# Autodesk Inventor assembly: Cottini lamp2
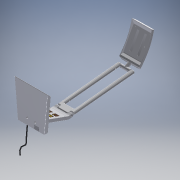
[picture p0: Inventor's stored thumbnail of the model, 180x180]
Saved by Autodesk Inventor 2016 (Build 200138000, 138)
## iProperties
Created: 2017-09-04
Part Number: Cottini lamp2
Document SubType Name: Assembly
Designer: Davide
Author: Davide
## Documents named in this file (22)
- C:\Users\Davide\Documents\Inventor\Cottini Lamp\Cottini lamp2.iam
- C:\Users\Davide\Documents\Inventor\Cottini Lamp\base bella.ipt
- C:\Users\Davide\Documents\Inventor\Cottini Lamp\perno bello.ipt
- C:\Users\Davide\Documents\Inventor\Cottini Lamp\USB Case.ipt
- C:\Users\Davide\Documents\Inventor\Cottini Lamp\cable.ipt
- C:\Users\Davide\Documents\Inventor\Cottini Lamp\tavolo.ipt
- C:\Users\Davide\Documents\Inventor\Cottini Lamp\primoblocco1.ipt
- C:\Users\Davide\Documents\Inventor\Cottini Lamp\placca.ipt
- C:\Users\Davide\Documents\Inventor\Content Center Files\R2016\en-US\AS 1427(03)\AS 1427 - M2 x 5(1).ipt
- C:\Users\Davide\Documents\Inventor\Cottini Lamp\Open_Book.ipt
- C:\Users\Davide\Documents\Inventor\Cottini Lamp\proiettore bello1.ipt
- C:\Users\Davide\Documents\Inventor\Cottini Lamp\astabella_lunga.ipt
- C:\Users\Davide\Documents\Inventor\Cottini Lamp\astabella_bassa.ipt
- C:\Users\Davide\Documents\Inventor\Content Center Files\R2016\en-US\AS 1112 (2)\AS 1112 - M4  Type 5.ipt
- C:\Users\Davide\Documents\Inventor\Content Center Files\R2016\en-US\AS 1427(05)\AS 1427 - M4 x 25(5) II.ipt
- C:\Users\Davide\Documents\Inventor\Content Center Files\R2016\en-US\AS 1420\AS 1420 - 1973 - M4 x 25.ipt
- C:\Users\Davide\Documents\Inventor\Content Center Files\R2016\en-US\AS 1112 (4)\AS 1112 - M4(2).ipt
- C:\Users\Davide\Documents\Inventor\Cottini Lamp\button1.ipt
- C:\Users\Davide\Documents\Inventor\Cottini Lamp\button2.ipt
- C:\Users\Davide\Documents\Inventor\Cottini Lamp\button3.ipt
- C:\Users\Davide\Documents\Inventor\Cottini Lamp\button4.ipt
- C:\Users\Davide\Documents\Inventor\Cottini Lamp\coperchietto.ipt
## Components (34 placed, 21 different names)
1. base bella:1 — Mate:47, Mate:49, Mate:50, Mate:51, Mate:79, Flush:1, Mate:80, Mate:94, Mate:95, Mate:96, Mate:110, Mate:112, Mate:209, Mate:210, Mate:211
2. perno bello:1 — Mate:147, Mate:148, Mate:153, Mate:173, Mate:175, Mate:178, Mate:180, Mate:182, Mate:183
3. USB Case:1 — Mate:79, Flush:1, Mate:80
4. cable:1 — Mate:112
5. tavolo:1 — Mate:94, Mate:146
6. primoblocco1:1 — Mate:95, Mate:96, Mate:138, Mate:139, Mate:155, Mate:160, Mate:161, Mate:164, Mate:165, Mate:166, Mate:167, Mate:188, Mate:207, Mate:208
7. placca:1 — Flush:6, Flush:7, Mate:192, Flush:12, Mate:199, Mate:200, Flush:13, Mate:201, Mate:202, Flush:14, Mate:203, Mate:204, Flush:15, Mate:205, Mate:206, Mate:207, Mate:208
8. Open_Book:1 — Mate:146
9. proiettore bello1:1 — Mate:147, Mate:148
10. astabella_lunga:1 — Mate:149, Mate:150, Mate:151, Mate:153, Mate:169, Mate:170, Mate:171, Mate:172
11. astabella_bassa:1 — Mate:149, Mate:150, Mate:151, Mate:155, Mate:168, Mate:185, Mate:187
12. button1:1 — Flush:12, Mate:199, Mate:200
13. button2:1 — Flush:13, Mate:201, Mate:202
14. button3:1 — Flush:14, Mate:203, Mate:204
15. button4:1 — Flush:15, Mate:205, Mate:206
16. coperchietto:1 — Mate:209, Mate:210, Mate:211, Mate:212, Mate:213, Flush:16, Flush:17
17. AS 1427 H - Metric M4 x 25:1 — Mate:47, Mate:51, Mate:158
18. AS 1427 H - Metric M4 x 25:2 — Mate:49, Mate:50, Mate:159
19. AS 1427 - Metric M2 x 5:2 — Mate:138, Flush:6, Mate:192
20. AS 1427 - Metric M2 x 5:3 — Mate:188
21. AS 1427 - Metric M2 x 5:6 — Mate:213, Flush:16
22. AS 1427 - Metric M2 x 5:7 — Mate:212, Flush:17
23. AS 1112 (2) - Metric M4  Type 5:1 — Mate:158, Mate:161
24. AS 1112 (2) - Metric M4  Type 5:2 — Mate:159, Mate:160
25. AS 1427 - Metric M2 x 5:4
26. AS 1427 - Metric M2 x 5:5 — Mate:139, Flush:7
27. AS 1420 - Metric M4 x 25:1 — Mate:164, Mate:167, Mate:184
28. AS 1420 - Metric M4 x 25:2 — Mate:165, Mate:166, Mate:168, Mate:186
29. AS 1420 - Metric M4 x 25:3 — Mate:169, Mate:170, Mate:175, Mate:178, Mate:179
30. AS 1420 - Metric M4 x 25:4 — Mate:171, Mate:172, Mate:173, Mate:181, Mate:182
31. AS 1112 (4) - Metric M4:1 — Mate:179, Mate:180
32. AS 1112 (4) - Metric M4:2 — Mate:181, Mate:183
33. AS 1112 (4) - Metric M4:3 — Mate:184, Mate:185
34. AS 1112 (4) - Metric M4:4 — Mate:186, Mate:187
## Relationships (74: Mate 65, Flush 9)
- Mate:47: base bella:1 ↔ AS 1427 H - Metric M4 x 25:1
- Mate:49: base bella:1 ↔ AS 1427 H - Metric M4 x 25:2
- Mate:50: base bella:1 ↔ AS 1427 H - Metric M4 x 25:2
- Mate:51: base bella:1 ↔ AS 1427 H - Metric M4 x 25:1
- Mate:79: base bella:1 ↔ USB Case:1
- Flush:1 (1 mm): base bella:1 ↔ USB Case:1
- Mate:80: base bella:1 ↔ USB Case:1
- Mate:94: base bella:1 ↔ tavolo:1
- Mate:95: base bella:1 ↔ primoblocco1:1
- Mate:96: base bella:1 ↔ primoblocco1:1
- Mate:110: base bella:1
- Mate:112: base bella:1 ↔ cable:1
- Mate:138: primoblocco1:1 ↔ AS 1427 - Metric M2 x 5:2
- Mate:139: primoblocco1:1 ↔ AS 1427 - Metric M2 x 5:5
- Flush:6: placca:1 ↔ AS 1427 - Metric M2 x 5:2
- Flush:7: placca:1 ↔ AS 1427 - Metric M2 x 5:5
- Mate:146: tavolo:1 ↔ Open_Book:1
- Mate:147: perno bello:1 ↔ proiettore bello1:1
- Mate:148: perno bello:1 ↔ proiettore bello1:1
- Mate:149: astabella_lunga:1 ↔ astabella_bassa:1
- Mate:150: astabella_lunga:1 ↔ astabella_bassa:1
- Mate:151: astabella_lunga:1 ↔ astabella_bassa:1
- Mate:153: perno bello:1 ↔ astabella_lunga:1
- Mate:155: primoblocco1:1 ↔ astabella_bassa:1
- Mate:158: AS 1427 H - Metric M4 x 25:1 ↔ AS 1112 (2) - Metric M4  Type 5:1
- Mate:159: AS 1427 H - Metric M4 x 25:2 ↔ AS 1112 (2) - Metric M4  Type 5:2
- Mate:160: primoblocco1:1 ↔ AS 1112 (2) - Metric M4  Type 5:2
- Mate:161: primoblocco1:1 ↔ AS 1112 (2) - Metric M4  Type 5:1
- Mate:164: primoblocco1:1 ↔ AS 1420 - Metric M4 x 25:1
- Mate:165: primoblocco1:1 ↔ AS 1420 - Metric M4 x 25:2
- Mate:166 (-4 mm): primoblocco1:1 ↔ AS 1420 - Metric M4 x 25:2
- Mate:167 (-4 mm): primoblocco1:1 ↔ AS 1420 - Metric M4 x 25:1
- Mate:168: astabella_bassa:1 ↔ AS 1420 - Metric M4 x 25:2
- Mate:169: astabella_lunga:1 ↔ AS 1420 - Metric M4 x 25:3
- Mate:170 (-4 mm): astabella_lunga:1 ↔ AS 1420 - Metric M4 x 25:3
- Mate:171: astabella_lunga:1 ↔ AS 1420 - Metric M4 x 25:4
- Mate:172 (-4 mm): astabella_lunga:1 ↔ AS 1420 - Metric M4 x 25:4
- Mate:173: perno bello:1 ↔ AS 1420 - Metric M4 x 25:4
- Mate:175: perno bello:1 ↔ AS 1420 - Metric M4 x 25:3
- [Mate]: AS 1420 - Metric M4 x 25:4 ↔ AS 1112 (4) - Metric M4:2
- [Mate]: perno bello:1 ↔ AS 1112 (4) - Metric M4:2
- Mate:178: perno bello:1 ↔ AS 1420 - Metric M4 x 25:3
- Mate:179: AS 1420 - Metric M4 x 25:3 ↔ AS 1112 (4) - Metric M4:1
- Mate:180: perno bello:1 ↔ AS 1112 (4) - Metric M4:1
- Mate:181: AS 1420 - Metric M4 x 25:4 ↔ AS 1112 (4) - Metric M4:2
- Mate:182: perno bello:1 ↔ AS 1420 - Metric M4 x 25:4
- Mate:183: perno bello:1 ↔ AS 1112 (4) - Metric M4:2
- Mate:184: AS 1420 - Metric M4 x 25:1 ↔ AS 1112 (4) - Metric M4:3
- Mate:185: astabella_bassa:1 ↔ AS 1112 (4) - Metric M4:3
- Mate:186: AS 1420 - Metric M4 x 25:2 ↔ AS 1112 (4) - Metric M4:4
- Mate:187: astabella_bassa:1 ↔ AS 1112 (4) - Metric M4:4
- Mate:188: primoblocco1:1 ↔ AS 1427 - Metric M2 x 5:3
- Mate:192: placca:1 ↔ AS 1427 - Metric M2 x 5:2
- Flush:12: placca:1 ↔ button1:1
- Mate:199: placca:1 ↔ button1:1
- Mate:200: placca:1 ↔ button1:1
- Flush:13: placca:1 ↔ button2:1
- Mate:201: placca:1 ↔ button2:1
- Mate:202: placca:1 ↔ button2:1
- Flush:14: placca:1 ↔ button3:1
- Mate:203: placca:1 ↔ button3:1
- Mate:204: placca:1 ↔ button3:1
- Flush:15: placca:1 ↔ button4:1
- Mate:205: placca:1 ↔ button4:1
- Mate:206: placca:1 ↔ button4:1
- Mate:207: primoblocco1:1 ↔ placca:1
- Mate:208: primoblocco1:1 ↔ placca:1
- Mate:209: base bella:1 ↔ coperchietto:1
- Mate:210: base bella:1 ↔ coperchietto:1
- Mate:211: base bella:1 ↔ coperchietto:1
- Mate:212: coperchietto:1 ↔ AS 1427 - Metric M2 x 5:7
- Mate:213: coperchietto:1 ↔ AS 1427 - Metric M2 x 5:6
- Flush:16: coperchietto:1 ↔ AS 1427 - Metric M2 x 5:6
- Flush:17: coperchietto:1 ↔ AS 1427 - Metric M2 x 5:7
